# Autodesk Inventor assembly: Przekładnie pasowe synchroniczne
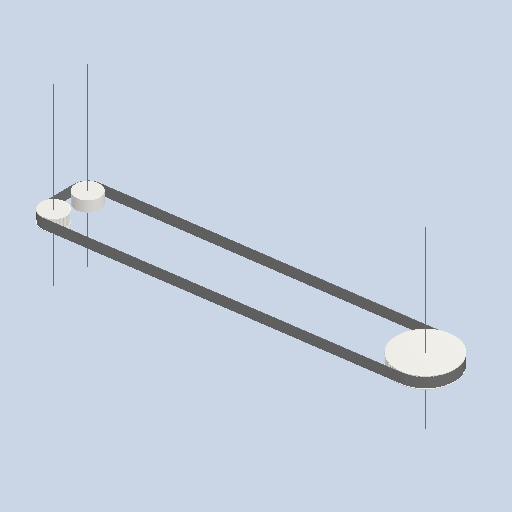
[picture p0: Inventor's stored thumbnail of the model, 512x512]
Saved by Autodesk Inventor 2023 (Build 270158000, 158)
## iProperties
ClientObjectVersion: 1
Created: 2023-04-25
Part Number: Przekładnie pasowe synchroniczne
Document SubType Name: Assembly
Designer: krzys
Author: krzys
## Documents named in this file (5)
- C:\Users\krzys\Documents\GitHub\Manipulator-Inventor\Manipulator\Design Accelerator\Przekładnie pasowe synchroniczne2.iam
- C:\Users\krzys\Documents\GitHub\Manipulator-Inventor\Manipulator\Design Accelerator\Pas synchroniczny2.ipt
- C:\Users\krzys\Documents\GitHub\Manipulator-Inventor\Manipulator\Design Accelerator\Synchroniczne koło pasowe12.ipt
- C:\Users\krzys\Documents\GitHub\Manipulator-Inventor\Manipulator\Design Accelerator\Synchroniczne koło pasowe22.ipt
- C:\Users\krzys\Documents\GitHub\Manipulator-Inventor\Manipulator\Design Accelerator\Koło pasowe zwykłe12.ipt
## Components (4 placed, 4 different names)
1. Pas synchroniczny:1 — Równoległe:1, Zestawiające:1, Zestawiające:2, Równoległe:2, Zestawiające:3, Zestawiające:4, Równoległe:3, Zestawiające:5
2. Synchroniczne koło pasowe1:1 — Równoległe:1, Zestawiające:1, Zestawiające:2, Obrót:1, Obrót:2
3. Synchroniczne koło pasowe2:1 — Równoległe:2, Zestawiające:3, Obrót:1, Zestawiające:4
4. Koło pasowe zwykłe1:1 — Równoległe:3, Zestawiające:5, Obrót:2
## Relationships (10: Mate 5, Flush 3, RelateRotation 2)
- Równoległe:1 [Flush]: Pas synchroniczny:1 ↔ Synchroniczne koło pasowe1:1
- Zestawiające:1 [Mate]: Pas synchroniczny:1 ↔ Synchroniczne koło pasowe1:1
- Zestawiające:2 [Mate]: Pas synchroniczny:1 ↔ Synchroniczne koło pasowe1:1
- Równoległe:2 [Flush]: Pas synchroniczny:1 ↔ Synchroniczne koło pasowe2:1
- Zestawiające:3 [Mate]: Pas synchroniczny:1 ↔ Synchroniczne koło pasowe2:1
- Obrót:1 [RelateRotation] (0.4167 ul): Synchroniczne koło pasowe1:1 ↔ Synchroniczne koło pasowe2:1
- Zestawiające:4 [Mate]: Pas synchroniczny:1 ↔ Synchroniczne koło pasowe2:1
- Równoległe:3 [Flush]: Pas synchroniczny:1 ↔ Koło pasowe zwykłe1:1
- Zestawiające:5 [Mate]: Pas synchroniczny:1 ↔ Koło pasowe zwykłe1:1
- Obrót:2 [RelateRotation] (0.4545 ul): Synchroniczne koło pasowe1:1 ↔ Koło pasowe zwykłe1:1
